# Autodesk Inventor assembly: diagonalstretcher
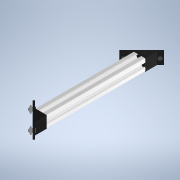
[picture p0: Inventor's stored thumbnail of the model, 180x180]
Saved by Autodesk Inventor 2020.2 (Build 242310000, 310)
## iProperties
Created: 2020-07-25
Part Number: diagonalstretcher
Document SubType Name: Assembly
Designer: JK
Author: JK
## Documents named in this file (3)
- C:\Users\JK\Documents\Inventor\Mesa\diagonalstretcher.iam
- C:\Users\JK\Documents\Inventor\Mesa\30x30x250.ipt
- C:\Users\JK\Documents\Inventor\Mesa\45degreebracketassembly.iam
## Components (3 placed, 2 different names)
1. 30x30x250:1 — Mate:1, Mate:2, Mate:3, Flush:1, Mate:4, Flush:2
2. 45degreebracketassembly:1 [sub-assembly] — Mate:1, Mate:3, Flush:1
3. 45degreebracketassembly:4 [sub-assembly] — Mate:2, Mate:4, Flush:2
## Relationships (6: Mate 4, Flush 2)
- Mate:1: 30x30x250:1 ↔ 45degreebracketassembly:1
- Mate:2: 30x30x250:1 ↔ 45degreebracketassembly:4
- Mate:3: 30x30x250:1 ↔ 45degreebracketassembly:1
- Flush:1: 30x30x250:1 ↔ 45degreebracketassembly:1
- Mate:4: 30x30x250:1 ↔ 45degreebracketassembly:4
- Flush:2: 30x30x250:1 ↔ 45degreebracketassembly:4
